# Autodesk Inventor assembly: Ejes
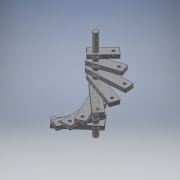
[picture p0: Inventor's stored thumbnail of the model, 180x180]
Saved by Autodesk Inventor 2019 (Build 230136000, 136)
## iProperties
Created: 2019-09-30
Part Number: Ejes
Document SubType Name: Assembly
Designer: Domenico
Author: Domenico
## Documents named in this file (7)
- C:\Users\Domenico\Documents\Inventor\Proyecto plantea\Ejes.iam
- C:\Users\Domenico\Documents\Inventor\Proyecto plantea\Ejes\Design Accelerator\Eje Principal - Interno.iam
- C:\Users\Domenico\Documents\Inventor\Proyecto plantea\Separador_grande.ipt
- C:\Users\Domenico\Documents\Inventor\Proyecto plantea\Separador_pequeño.ipt
- C:\Users\Domenico\Documents\Inventor\Proyecto plantea\Transmisor_grande.ipt
- C:\Users\Domenico\Documents\Inventor\Proyecto plantea\Transmisor_mediano.ipt
- C:\Users\Domenico\Documents\Inventor\Proyecto plantea\Transmisor_pequeño.ipt
## Components (19 placed, 6 different names)
1. Eje Principal - Interno:1 [sub-assembly] — Mate:1, Mate:2, Mate:3, Mate:4, Mate:5, Mate:6, Mate:7, Mate:8, Mate:9, Flush:1, Mate:10, Mate:13, Mate:14, Mate:15, Mate:16, Mate:17, Mate:28, Mate:31, Mate:34
2. Separador_pequeño:1 — Mate:7, Mate:30, Mate:35
3. Separador_pequeño:2 — Mate:3, Mate:25, Mate:26
4. Separador_pequeño:3 — Mate:2, Mate:12, Mate:18
5. Separador_pequeño:4 — Mate:8, Mate:19, Mate:20
6. Separador_pequeño:5 — Mate:9, Mate:36, Mate:37
7. Separador_pequeño:6 — Mate:6, Mate:21, Mate:22
8. Separador_pequeño:7 — Mate:5, Mate:23, Mate:24
9. Separador_pequeño:8 — Mate:4, Mate:27, Mate:29
10. Separador_grande:2 — Mate:1, Flush:1, Mate:11
11. Transmisor_grande:1 — Mate:14, Mate:20, Mate:21
12. Transmisor_grande:2 — Mate:16, Mate:24, Mate:25
13. Transmisor_grande:3 — Mate:17, Mate:26, Mate:27
14. Transmisor_grande:4 — Mate:28, Mate:29, Mate:30
15. Transmisor_grande:5 — Mate:15, Mate:22, Mate:23
16. Transmisor_grande:6 — Mate:10, Mate:11, Mate:12
17. Transmisor_grande:7 — Mate:13, Mate:18, Mate:19
18. Transmisor_mediano:1 — Mate:34, Mate:35, Mate:36
19. Transmisor_pequeño:1 — Mate:31, Mate:37
## Relationships (36: Mate 35, Flush 1)
- Mate:1: Eje Principal - Interno:1 ↔ Separador_grande:2
- Mate:2: Eje Principal - Interno:1 ↔ Separador_pequeño:3
- Mate:3: Eje Principal - Interno:1 ↔ Separador_pequeño:2
- Mate:4: Eje Principal - Interno:1 ↔ Separador_pequeño:8
- Mate:5: Eje Principal - Interno:1 ↔ Separador_pequeño:7
- Mate:6: Eje Principal - Interno:1 ↔ Separador_pequeño:6
- Mate:7: Eje Principal - Interno:1 ↔ Separador_pequeño:1
- Mate:8: Eje Principal - Interno:1 ↔ Separador_pequeño:4
- Mate:9: Eje Principal - Interno:1 ↔ Separador_pequeño:5
- Flush:1 (10 mm): Eje Principal - Interno:1 ↔ Separador_grande:2
- Mate:10: Eje Principal - Interno:1 ↔ Transmisor_grande:6
- Mate:11 (4.5 mm): Separador_grande:2 ↔ Transmisor_grande:6
- Mate:12 (4.5 mm): Separador_pequeño:3 ↔ Transmisor_grande:6
- Mate:13: Eje Principal - Interno:1 ↔ Transmisor_grande:7
- Mate:14: Eje Principal - Interno:1 ↔ Transmisor_grande:1
- Mate:15: Eje Principal - Interno:1 ↔ Transmisor_grande:5
- Mate:16: Eje Principal - Interno:1 ↔ Transmisor_grande:2
- Mate:17: Eje Principal - Interno:1 ↔ Transmisor_grande:3
- Mate:18 (4.5 mm): Separador_pequeño:3 ↔ Transmisor_grande:7
- Mate:19 (4.5 mm): Separador_pequeño:4 ↔ Transmisor_grande:7
- Mate:20 (4.5 mm): Separador_pequeño:4 ↔ Transmisor_grande:1
- Mate:21 (4.5 mm): Separador_pequeño:6 ↔ Transmisor_grande:1
- Mate:22 (4.5 mm): Separador_pequeño:6 ↔ Transmisor_grande:5
- Mate:23 (4.5 mm): Separador_pequeño:7 ↔ Transmisor_grande:5
- Mate:24 (4.5 mm): Separador_pequeño:7 ↔ Transmisor_grande:2
- Mate:25 (4.5 mm): Separador_pequeño:2 ↔ Transmisor_grande:2
- Mate:26 (4.5 mm): Separador_pequeño:2 ↔ Transmisor_grande:3
- Mate:27 (4.5 mm): Separador_pequeño:8 ↔ Transmisor_grande:3
- Mate:28: Eje Principal - Interno:1 ↔ Transmisor_grande:4
- Mate:29 (4.5 mm): Separador_pequeño:8 ↔ Transmisor_grande:4
- Mate:30 (4.5 mm): Separador_pequeño:1 ↔ Transmisor_grande:4
- Mate:31: Eje Principal - Interno:1 ↔ Transmisor_pequeño:1
- Mate:34: Eje Principal - Interno:1 ↔ Transmisor_mediano:1
- Mate:35 (4.5 mm): Separador_pequeño:1 ↔ Transmisor_mediano:1
- Mate:36 (4.5 mm): Separador_pequeño:5 ↔ Transmisor_mediano:1
- Mate:37 (4.5 mm): Separador_pequeño:5 ↔ Transmisor_pequeño:1
## Named parameters: diametro_externo = 25.4 mm, diametro_interno = 23.4 mm, ancho_de_cara = 4.5 mm
